# Autodesk Inventor assembly: DD_KVD_001
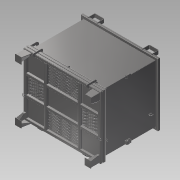
[picture p0: Inventor's stored thumbnail of the model, 180x180]
Saved by Autodesk Inventor 2017.3 (Build 213256000, 256)
## iProperties
Created: 2023-12-08
Part Number: DD_KVD_001
Document SubType Name: Assembly
Designer: Darena
Author: Darena
## Documents named in this file (6)
- D:\2_Darena\1_Soukrome\02_Inventor soukromé\Dílna RAKO3\Záhora\Pivovar KONTEJNER\S výklopným dnem\DD_KVD_001\DD_KVD_001.iam
- D:\2_Darena\1_Soukrome\02_Inventor soukromé\Dílna RAKO3\Záhora\Pivovar KONTEJNER\S výklopným dnem\DD_KVD_001\DD_KVD_003.iam
- D:\2_Darena\1_Soukrome\02_Inventor soukromé\Dílna RAKO3\Záhora\Pivovar KONTEJNER\S výklopným dnem\DD_KVD_001\DD_KVD_002.iam
- D:\2_Darena\1_Soukrome\02_Inventor soukromé\Dílna RAKO3\Záhora\Pivovar KONTEJNER\S výklopným dnem\DD_KVD_001\DD_KVD_003_10_B.ipt
- D:\2_Darena\1_Soukrome\02_Inventor soukromé\Dílna RAKO3\Záhora\Pivovar KONTEJNER\S výklopným dnem\DD_KVD_001\DD_KVD_003_10_C.ipt
- D:\2_Darena\1_Soukrome\02_Inventor soukromé\Dílna RAKO3\Záhora\Pivovar KONTEJNER\S výklopným dnem\DD_KVD_001\DD_KVD_003_10_D.ipt
## Components (8 placed, 5 different names)
1. DD_KVD_002:1 [sub-assembly] — Proti sobě:3, Vložit:1, Vložit:2, Vložit:3, Vložit:5, ZAVŘENO, Stejný směr:1, Stejný směr:2, Stejný směr:3
2. DD_KVD_003:1 [sub-assembly] — Proti sobě:1, Proti sobě:3, PANT, ZAVŘENO
3. DD_KVD_003_10_B:1 — Vložit:1, Vložit:4, PANT
4. DD_KVD_003_10_C:1 — Vložit:5
5. DD_KVD_003_10_D:1 — Vložit:6
6. DD_KVD_003_10_B:2 — Vložit:2, Vložit:6
7. DD_KVD_003_10_C:2 — Vložit:3
8. DD_KVD_003_10_D:2 — Vložit:4
## Relationships (13: Insert 6, Mate 4, Flush 3)
- Proti sobě:1 [Mate]: DD_KVD_003:1
- Proti sobě:3 [Mate]: DD_KVD_002:1 ↔ DD_KVD_003:1
- Vložit:1 [Insert]: DD_KVD_002:1 ↔ DD_KVD_003_10_B:1
- Vložit:2 [Insert]: DD_KVD_002:1 ↔ DD_KVD_003_10_B:2
- Vložit:3 [Insert]: DD_KVD_002:1 ↔ DD_KVD_003_10_C:2
- Vložit:4 [Insert]: DD_KVD_003_10_B:1 ↔ DD_KVD_003_10_D:2
- Vložit:5 [Insert]: DD_KVD_002:1 ↔ DD_KVD_003_10_C:1
- Vložit:6 [Insert]: DD_KVD_003_10_D:1 ↔ DD_KVD_003_10_B:2
- PANT [Mate]: DD_KVD_003:1 ↔ DD_KVD_003_10_B:1
- ZAVŘENO [Mate]: DD_KVD_002:1 ↔ DD_KVD_003:1
- Stejný směr:1 [Flush]: DD_KVD_002:1
- Stejný směr:2 [Flush]: DD_KVD_002:1
- Stejný směr:3 [Flush]: DD_KVD_002:1
